# Autodesk Inventor assembly: TEST
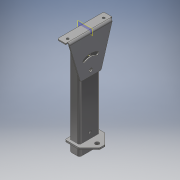
[picture p0: Inventor's stored thumbnail of the model, 180x180]
Saved by Autodesk Inventor 2017 (Build 210142000, 142)
## iProperties
Created: 2017-01-07
Part Number: TEST
Document SubType Name: Assembly
Designer: bramp
RuleStatus: InUse
Author: bramp
## Documents named in this file (6)
- D:\Gebruikers\bramp\Documents\Test\InventorBram\TEST.iam
- D:\Gebruikers\bramp\Documents\Test\InventorBram\Cprofiel.ipt
- D:\Gebruikers\bramp\Documents\Test\InventorBram\U schuif.ipt
- D:\Gebruikers\bramp\Documents\Test\InventorBram\90-01-0000.ipt
- D:\Gebruikers\bramp\Documents\Test\InventorBram\90-02-0000.ipt
- D:\Gebruikers\bramp\Documents\Test\InventorBram\90-03-0000.ipt
## Components (6 placed, 5 different names)
1. Cprofiel:1 — Mate:1, Mate:2, Mate:3, Mate:4, Mate:5, Mate:6, Mate:8
2. U schuif:1 — Mate:1, Mate:14, Mate:2, Mate:7, Mate:9, Mate:10, Mate:11, Mate:12, Mate:13
3. 90-01-0000:1 — Mate:3, Mate:4, Mate:5, Angle:1, Mate:14
4. 90-02-0000:1 — Mate:6, Mate:7, Angle:1
5. 90-03-0000:1 — Mate:9, Mate:10, Mate:11
6. 90-03-0000:2 — Mate:8, Mate:12, Mate:13
## Relationships (15: Mate 14, Angle 1)
- Mate:1 (1 mm): Cprofiel:1 ↔ U schuif:1
- Mate:14 (-305 mm): U schuif:1 ↔ 90-01-0000:1
- Mate:2: Cprofiel:1 ↔ U schuif:1
- Mate:3: Cprofiel:1 ↔ 90-01-0000:1
- Mate:4 (0.5 mm): Cprofiel:1 ↔ 90-01-0000:1
- Mate:5 (0.5 mm): Cprofiel:1 ↔ 90-01-0000:1
- Mate:6 (4 mm): Cprofiel:1 ↔ 90-02-0000:1
- Mate:7: U schuif:1 ↔ 90-02-0000:1
- Angle:1 (0 deg): 90-01-0000:1 ↔ 90-02-0000:1
- Mate:8: Cprofiel:1 ↔ 90-03-0000:2
- Mate:9: U schuif:1 ↔ 90-03-0000:1
- Mate:10: U schuif:1 ↔ 90-03-0000:1
- Mate:11: U schuif:1 ↔ 90-03-0000:1
- Mate:12: U schuif:1 ↔ 90-03-0000:2
- Mate:13: U schuif:1 ↔ 90-03-0000:2
## Named parameters: HoogtBovenplaat = -305 mm, HoekScharnierplaat = 0 deg, HoogteGatenTravers = 18.5 mm
